# Autodesk Inventor assembly: Bottom Assembly--v1
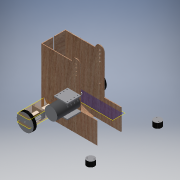
[picture p0: Inventor's stored thumbnail of the model, 180x180]
Saved by Autodesk Inventor 2019 (Build 230136000, 136)
## iProperties
Created: 2019-01-29
Part Number: Bottom Assembly--v1
Document SubType Name: Assembly
Designer: scigu
Author: scigu
## Documents named in this file (7)
- C:\Users\scigu\Documents\School 18-19\SeCon\Chassis\Bottom Assembly--v1.iam
- C:\Users\scigu\Documents\School 18-19\SeCon\Chassis\Small Motor.ipt
- C:\Users\scigu\Documents\School 18-19\SeCon\Chassis\Wheel.ipt
- C:\Users\scigu\Documents\School 18-19\SeCon\Chassis\Caster.ipt
- C:\Users\scigu\Documents\School 18-19\SeCon\Intake\Wall--v3_Left.ipt
- C:\Users\scigu\Documents\School 18-19\SeCon\Intake\Wall--v3_Right.ipt
- C:\Users\scigu\Documents\School 18-19\SeCon\Chassis\Big Motor.ipt
## Components (9 placed, 6 different names)
1. Small Motor:1 — Mate:1, Mate:2, Flush:2, Insert:2, Tangent:8, Mate:5
2. Small Motor:2 — Flush:1, Mate:2, Flush:2, Insert:1, Flush:3, Tangent:7, Mate:3, Angle:2, Flush:10
3. Wheel:1 — Insert:2, Tangent:10
4. Wheel:2 — Insert:1, Tangent:1, Tangent:2, Tangent:9, Tangent:11
5. Caster:1 — Tangent:5, Tangent:6, Tangent:8
6. Caster:2 — Tangent:3, Tangent:4, Tangent:7
7. Wall--v3_Left:1 — Mate:3, Mate:4, Tangent:9, Mate:7
8. Wall--v3_Right:1 — Mate:5, Mate:6, Tangent:10, Flush:12
9. Big Motor:1 — Mate:7, Angle:1
## Relationships (34: Flush 12, Tangent 11, Mate 7, Insert 2, Angle 2)
- Flush:1 (-111.125 mm): Small Motor:2
- Mate:1 (-111.125 mm): Small Motor:1
- Mate:2: Small Motor:1 ↔ Small Motor:2
- Flush:2: Small Motor:1 ↔ Small Motor:2
- Insert:1 (2.54 mm): Small Motor:2 ↔ Wheel:2
- Insert:2 (2.54 mm): Small Motor:1 ↔ Wheel:1
- Tangent:1: Wheel:2
- Tangent:2 (3.175 mm): Wheel:2
- Flush:3 (-43.0022 mm): Small Motor:2
- Tangent:3: Caster:2
- Tangent:4 (-225.425 mm): Caster:2
- Tangent:5: Caster:1
- Tangent:6 (-225.425 mm): Caster:1
- Tangent:7: Small Motor:2 ↔ Caster:2
- Tangent:8: Small Motor:1 ↔ Caster:1
- Mate:3: Small Motor:2 ↔ Wall--v3_Left:1
- Mate:4: Wall--v3_Left:1
- Tangent:9: Wheel:2 ↔ Wall--v3_Left:1
- Mate:5: Small Motor:1 ↔ Wall--v3_Right:1
- Mate:6: Wall--v3_Right:1
- Tangent:10: Wheel:1 ↔ Wall--v3_Right:1
- Mate:7: Wall--v3_Left:1 ↔ Big Motor:1
- Angle:1 (180 deg): Big Motor:1
- Flush:4
- Flush:5
- Flush:6 (114.3 mm)
- Flush:7 (-114.3 mm)
- Flush:8 (228.6 mm)
- Flush:9 (279.4 mm)
- Angle:2 (0 deg): Small Motor:2
- Tangent:11: Wheel:2
- Flush:10: Small Motor:2
- Flush:11 (-22.5044 mm)
- Flush:12 (-50.8 mm): Wall--v3_Right:1
